# Autodesk Inventor assembly: SCSTR8-10
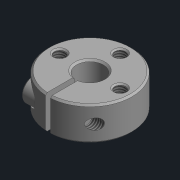
[picture p0: Inventor's stored thumbnail of the model, 180x180]
Saved by Autodesk Inventor 2022 (Build 260153000, 153)
## iProperties
Part Number: SCSTR8-10
Catalog Web Link: www.cadenas.de
Description: SCST, PSCST, SSCST, SCSTR, PSCSTR, SSCSTR-Shaft Collars - 3 Holes/3 Taps
Vendor: MISUMI
Document SubType Name: Assembly
Designer: partserver
Manufacturer: MISUMI
Mass: 3.95691 g
Surface Area: 27.1551 cm^2
Volume: 3.95691 cm^3
Density: 1 g/cm^3
Category: PARTsolutions
Company: MISUMI
PSOL_IDENT_0: {$CADENAS_DATA\23d-libs\misumi\metric\03_set_collars\scst_asmtab.prj},221 {VTYP=3D},{STYP=ASSTAB},{N
PSOL_IDENT_1: B=SCSTR8-10},{LINA=SCSTR8-10},{NN=SCST, PSCST, SSCST, SCSTR, PSCSTR, SSCSTR},{DATE=30.06.2021 12:52:
PSOL_IDENT_2: 05},{GEOMDATE=30.10.2015 01:45:58},{VERSION=},{LINEID=50},{WBVAR=TS,MAT,ST,BS},{WBNUMERIC=BS}  {NB=S
PSOL_IDENT_3: CSTR8-10},{LINA=SCSTR8-10},{KT=DUMMY},{PN=SCSTR8-10},{TYPE=SCSTR},{TS=3T},{TSALG= '3H' , '3-Hole' , '
PSOL_IDENT_4: 3T' , '3-Tapped' },{MAT=S45C},{ST=BO},{STALG= 'BO' , 'Black Oxide' , 'ENP' , 'Electroless Nickel Pla
PSOL_IDENT_5: ting' },{AC=Hex Socket Head Cap Screw 1 pc.},{ACMAT=4137 Alloy Steel},{D=8},{BS=10},{BALG= 8 , 10 },
PSOL_IDENT_6: {D1=25},{M=M4},{M3D=4},{DD=4.5},{R=3.75},{W=1.5},{X=8.0},{Y=5},{P=18},{C=0.5},{S=0.0},{M1=M4},{M13D=
PSOL_IDENT_7: 4},{L=12},{PPATH=scst/scst_templ.prj}
NB: SCSTR8-10
NN: SCST, PSCST, SSCST, SCSTR, PSCSTR, SSCSTR
NT: Shaft Collars - 3 Holes/3 Taps
NBSYN: $PN.
LINA: SCSTR8-10
CATALOG: Misumi
PN: SCSTR8-10
TS: 3-Tapped
MAT: 1045 Carbon Steel
ST: Black Oxide
AC: Hex Socket Head Cap Screw 1 pc.
ACMAT: 4137 Alloy Steel
D: 8
BS: 10
D1: 25
M: M4
DD: 4.5
R: 3.75
W: 1.5
X: 8
Y: 5
P: 18
C: 0.5
S: 0
M1: M4
SUPPLIER: MISUMI
ARTICLENO: SCSTR8-10
BOMINFO: SCSTR8-10
CREATOR: CADENAS GmbH
Title: SCSTR8-10
Author: Cadenas PARTsolutions
Comments: Shaft Collars - 3 Holes/3 Taps
## Documents named in this file (3)
- C:\Users\yuta0\Documents\GitHub\catchrobo_hardware\assy-scara\SCSTR8-10.iam
- C:\Users\yuta0\Documents\GitHub\catchrobo_hardware\assy-scara\SCSTR8-10b.ipt
- C:\Users\yuta0\Documents\GitHub\catchrobo_hardware\assy-scara\BOLT4-12.ipt
## Components (2 placed, 2 different names)
1. SCSTR8-10b:1 — to_bolt_XY@1 <-> to_cp_XY@2, to_bolt_Z@1 <-> to_cp_Z@2, to_bolt_YZ@1 <-> to_cp_YZ@2
2. BOLT4-12:1 — to_bolt_XY@1 <-> to_cp_XY@2, to_bolt_Z@1 <-> to_cp_Z@2, to_bolt_YZ@1 <-> to_cp_YZ@2
## Relationships (3: Mate 2, Angle 1)
- to_bolt_XY@1 <-> to_cp_XY@2 [Mate]: SCSTR8-10b:1 ↔ BOLT4-12:1
- to_bolt_Z@1 <-> to_cp_Z@2 [Mate]: SCSTR8-10b:1 ↔ BOLT4-12:1
- to_bolt_YZ@1 <-> to_cp_YZ@2 [Angle] (0 deg): SCSTR8-10b:1 ↔ BOLT4-12:1
